# Autodesk Inventor assembly: internalGearLock
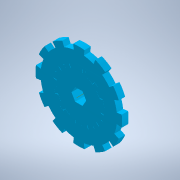
[picture p0: Inventor's stored thumbnail of the model, 180x180]
Saved by Autodesk Inventor 2021.2 (Build 252289000, 289)
## iProperties
Created: 2020-11-20
Part Number: internalGearLock
Document SubType Name: Assembly
Designer: robst
Author: robst
## Documents named in this file (3)
- C:\git\CAD-Development\robSteele\ShapeWays\TelescopeProjects\TelescopeMount\SplineLock\internalGearLock.iam
- C:\git\CAD-Development\robSteele\ShapeWays\TelescopeProjects\TelescopeMount\SplineLock\centerPartOfLock.ipt
- C:\git\CAD-Development\robSteele\ShapeWays\TelescopeProjects\TelescopeMount\SplineLock\outerPartOfLock.ipt
## Components (2 placed, 2 different names)
1. centerPartOfLock:1 — Insert:1
2. outerPartOfLock:1 — Insert:1
## Relationships (1: Insert 1)
- Insert:1: centerPartOfLock:1 ↔ outerPartOfLock:1
